# Autodesk Inventor assembly: Galileo Guide
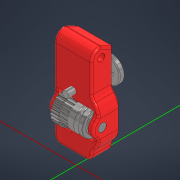
[picture p0: Inventor's stored thumbnail of the model, 180x180]
Saved by Autodesk Inventor 2022.2 (Build 262287010, 287A)
## iProperties
Created: 2022-03-15
Part Number: Galileo Guide
Document SubType Name: Assembly
Designer: sleib
Author: sleib
## Documents named in this file (5)
- C:\Users\sleib\Projekte\Voron-2\CAD\Inventor\Galileo Clockwork\Galileo Guide.iam
- C:\Users\sleib\Projekte\Voron-2\CAD\Inventor\Galileo Clockwork\Idler Guide.ipt
- C:\Users\sleib\Projekte\Voron-2\CAD\Inventor\Galileo Clockwork\Flygear.ipt
- C:\Users\sleib\Projekte\Voron-2\CAD\Inventor\Galileo Clockwork\Spring.ipt
- C:\Users\sleib\Projekte\Voron-2\CAD\Inventor\Galileo Clockwork\M3 Thumb Screw.ipt
## Components (4 placed, 4 different names)
1. Idler Guide:1 — Passend:1, Passend:2, Passend:3, Passend:4, Passend:5
2. Flygear:1 — Passend:1, Passend:2, Passend:3
3. Spring:1 — Passend:5, Passend:6
4. M3 Thumb Screw:1 — Passend:4, Passend:6
## Relationships (6: Mate 6)
- Passend:1 [Mate]: Idler Guide:1 ↔ Flygear:1
- Passend:2 [Mate]: Idler Guide:1 ↔ Flygear:1
- Passend:3 [Mate] (0.9 mm): Idler Guide:1 ↔ Flygear:1
- Passend:4 [Mate]: Idler Guide:1 ↔ M3 Thumb Screw:1
- Passend:5 [Mate]: Idler Guide:1 ↔ Spring:1
- Passend:6 [Mate]: Spring:1 ↔ M3 Thumb Screw:1
